# Autodesk Inventor assembly: Przekładnia
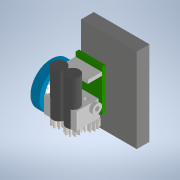
[picture p0: Inventor's stored thumbnail of the model, 180x180]
Saved by Autodesk Inventor 2022 (Build 260153000, 153)
## iProperties
Created: 2023-01-15
Part Number: Przekładnia
Document SubType Name: Assembly
Designer: komputer
Author: komputer
## Documents named in this file (13)
- D:\Inventor\NanoSumo\Przekładnia.iam
- D:\Inventor\NanoSumo\Moteur - Engrenage 3.ipt
- D:\Inventor\NanoSumo\silnik_2.ipt
- C:\Users\komputer\Desktop\Moteur - Axe engrenage.ipt
- D:\Inventor\NanoSumo\kokool.ipt
- D:\Inventor\NanoSumo\Przekładnia\Design Accelerator\Spur Gears2.iam
- D:\Inventor\NanoSumo\podłoga.ipt
- C:\Users\komputer\Desktop\Moteur - Engrenage 3_MIR1.ipt
- D:\Inventor\NanoSumo\Przekładnia\Design Accelerator\Spur Gears2_MIR1.iam
- D:\Inventor\NanoSumo\elem.ipt
- D:\PCBE.ipt
- D:\spod.ipt
- D:\pcb2.ipt
## Components (16 placed, 12 different names)
1. silnik_2:1 — Mate:21, Flush:6, Flush:7, Mate:30
2. silnik_2:3 — Mate:20, Flush:4, Flush:5, Mate:21, Flush:6, Flush:7, Flush:24
3. Moteur - Axe engrenage:2
4. Moteur - Axe engrenage:3
5. kokool:2 — Mate:26, Flush:11, Mate:42, Flush:26
6. Spur Gears:2 [sub-assembly] — Mate:30
7. podłoga:1 — Mate:20, Flush:4, Flush:5, Mate:24, Angle:1, Flush:11
8. Moteur - Engrenage 3:5 — Mate:42
9. Moteur - Engrenage 3_MIR1:1 — Mate:26
10. Spur Gears2_MIR1:1 [sub-assembly]
11. elem:1 — Flush:24, Mate:37, Mate:38, Flush:27, Flush:28
12. Moteur - Engrenage 3:6 — Mate:37, Mate:38, Mate:39
13. kokool:4 — Mate:39
14. spod:1 — Flush:26, Mate:43
15. PCBE:3 — Flush:27, Mate:43, Flush:28, Flush:29
16. pcb2:1 — Flush:29
## Relationships (21: Mate 10, Flush 10, Angle 1)
- Mate:20: silnik_2:3 ↔ podłoga:1
- Flush:4: silnik_2:3 ↔ podłoga:1
- Flush:5: silnik_2:3 ↔ podłoga:1
- Mate:21: silnik_2:1 ↔ silnik_2:3
- Flush:6: silnik_2:1 ↔ silnik_2:3
- Flush:7: silnik_2:1 ↔ silnik_2:3
- Mate:24: podłoga:1
- Angle:1 (0 deg): podłoga:1
- Mate:26: kokool:2 ↔ Moteur - Engrenage 3_MIR1:1
- Flush:11: kokool:2 ↔ podłoga:1
- Mate:30 (0.1 mm): silnik_2:1 ↔ Spur Gears:2
- Flush:24: silnik_2:3 ↔ elem:1
- Mate:37: elem:1 ↔ Moteur - Engrenage 3:6
- Mate:38 (0.3 mm): elem:1 ↔ Moteur - Engrenage 3:6
- Mate:39: Moteur - Engrenage 3:6 ↔ kokool:4
- Mate:42: kokool:2 ↔ Moteur - Engrenage 3:5
- Flush:26: kokool:2 ↔ spod:1
- Flush:27: elem:1 ↔ PCBE:3
- Mate:43 (3.5 mm): spod:1 ↔ PCBE:3
- Flush:28 (-0.6 mm): elem:1 ↔ PCBE:3
- Flush:29: PCBE:3 ↔ pcb2:1
